# Autodesk Inventor assembly: New_body
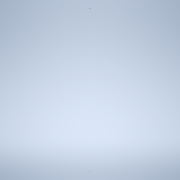
[picture p0: Inventor's stored thumbnail of the model, 180x180]
Saved by Autodesk Inventor 2022 (Build 260153000, 153)
## iProperties
Created: 2023-02-14
Part Number: New_body
Document SubType Name: Assembly
Designer: scott
Author: scott
## Documents named in this file (4)
- C:\Users\scott\OneDrive\Documents\Cat project\Git_repository\Flinders_OpenCat\CAD components\New_body.iam
- C:\Users\scott\OneDrive\Documents\Cat project\Git_repository\Flinders_OpenCat\CAD components\NybbleDIY\Imported Components\BellyPlate\BellyPlate.ipt
- C:\Users\scott\OneDrive\Documents\Cat project\Git_repository\Flinders_OpenCat\CAD components\Imported Components\pi_v6\pi_v6.ipt
- C:\Users\scott\OneDrive\Documents\Cat project\Git_repository\Flinders_OpenCat\CAD components\Imported Components\Nybble_y1\Nybble_y1.ipt
## Components (4 placed, 3 different names)
1. BellyPlate:1 — Mate:1
2. pi_v6:1
3. Nybble_y1:1 — Flush:1, Flush:2, Mate:1
4. Nybble_y1:2 — Flush:1, Flush:2
## Relationships (3: Flush 2, Mate 1)
- Flush:1: Nybble_y1:1 ↔ Nybble_y1:2
- Flush:2: Nybble_y1:1 ↔ Nybble_y1:2
- Mate:1 (7.5 mm): BellyPlate:1 ↔ Nybble_y1:1
